# Autodesk Inventor assembly: Bottom
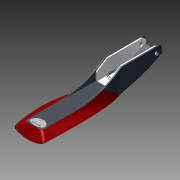
[picture p0: Inventor's stored thumbnail of the model, 180x180]
Saved by Autodesk Inventor 2011 (Build 150239000, 239)
## iProperties
Shininess: 64.0
Length Units: 11272
Angle Units: 11279
Time Units: 11290
Mass Units: 11286
Length Display Precision: 3
Angle Display Precision: 2
Compacted: True
Part Number: Bottom
Document SubType Name: Assembly
Created: 2002-09-25
Designer: Autodesk, Inc.
Project: Inventor Samples
Mass: 81.8675 g
Surface Area: 309.342 cm^2
Volume: 50.0379 cm^3
Density: 1.63611 g/cm^3
Density: 0.0
Volumn: 0.0
Area: 0.0
PropertySet Name: Model Information
Control State: 0
Master: False
Checked Out: False
Author: Autodesk, Inc.
Revision Number: A
## Documents named in this file (6)
- C:\Users\Public\Documents\Autodesk\Inventor 2011\Samples\Models\Assemblies\Stapler\Components\Bottom.iam
- C:\Users\Public\Documents\Autodesk\Inventor 2011\Samples\Models\Assemblies\Stapler\Components\Bottom - Back.ipt
- C:\Users\Public\Documents\Autodesk\Inventor 2011\Samples\Models\Assemblies\Stapler\Components\Bottom - Front.ipt
- C:\Users\Public\Documents\Autodesk\Inventor 2011\Samples\Models\Assemblies\Stapler\Components\Lower Mount.ipt
- C:\Users\Public\Documents\Autodesk\Inventor 2011\Samples\Models\Assemblies\Stapler\Components\Spring.ipt
- C:\Users\Public\Documents\Autodesk\Inventor 2011\Samples\Models\Assemblies\Stapler\Components\Bottom - Anvil.ipt
## Components (5 placed, 5 different names)
1. Bottom - Back:1 — Mate:1, Mate:2, Flush:1, Flush:2, Flush:3, Flush:4, Mate:7, Mate:8
2. Bottom - Front:1 — Flush:3, Mate:7, Mate:8
3. Lower Mount:1 — Mate:1, Mate:2, Flush:1, Flush:2, Mate:3, Mate:4
4. Spring:1 — Mate:3, Mate:4
5. Bottom - Anvil:1 — Flush:4
## Relationships (10: Mate 6, Flush 4)
- Mate:1: Bottom - Back:1 ↔ Lower Mount:1
- Mate:2: Bottom - Back:1 ↔ Lower Mount:1
- Flush:1: Bottom - Back:1 ↔ Lower Mount:1
- Flush:2: Bottom - Back:1 ↔ Lower Mount:1
- Mate:3: Lower Mount:1 ↔ Spring:1
- Mate:4: Lower Mount:1 ↔ Spring:1
- Flush:3: Bottom - Back:1 ↔ Bottom - Front:1
- Flush:4: Bottom - Back:1 ↔ Bottom - Anvil:1
- Mate:7: Bottom - Back:1 ↔ Bottom - Front:1
- Mate:8: Bottom - Back:1 ↔ Bottom - Front:1
